# Autodesk Inventor assembly: base_ass_3
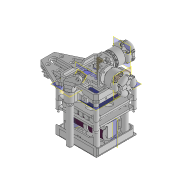
[picture p0: Inventor's stored thumbnail of the model, 180x180]
Saved by Autodesk Inventor 2020 (Build 240168000, 168)
## iProperties
Created: 2022-01-22
Part Number: base_ass_3
Document SubType Name: Assembly
Designer: Shuang Peng
Author: Shuang Peng
## Documents named in this file (18)
- D:\projects-3\soft module robot\hardware\diff module 3\base_ass_3.iam
- D:\projects-3\soft module robot\hardware\diff module 3\ext_shell_1.ipt
- D:\projects-3\soft module robot\hardware\diff module 3\brushless sub driver v1\brushless sub driver.iam
- D:\projects-3\soft module robot\hardware\diff module 3\pin_2_40.ipt
- D:\projects-3\soft module robot\hardware\diff module 3\ext_shell_2.ipt
- D:\projects-3\soft module robot\hardware\diff module 3\bridge_linker_1.ipt
- D:\projects-3\soft module robot\hardware\diff module 3\ext_shell_3.ipt
- D:\projects-3\soft module robot\hardware\diff module 3\bat_pack.iam
- D:\projects-3\soft module robot\hardware\diff module 3\ext_shell_top.ipt
- D:\projects-3\soft module robot\hardware\diff module 3\balancing_wheel_1.ipt
- D:\projects-3\soft module robot\hardware\diff module 3\balancing_wheel_2.ipt
- D:\projects-3\soft module robot\hardware\diff module 3\pin_6_40.ipt
- D:\projects-3\soft module robot\hardware\diff module 3\bearing_3_6_2.ipt
- D:\projects-3\soft module robot\hardware\diff module 3\c_roller_1.ipt
- D:\projects-3\soft module robot\hardware\diff module 3\tag.ipt
- D:\projects-3\soft module robot\hardware\diff module 3\wheel_pin_1.ipt
- D:\projects-3\soft module robot\hardware\diff module 3\pin_3_6.ipt
- D:\projects-3\soft module robot\hardware\diff module 3\2sr_ass_tmp.iam
## Components (27 placed, 17 different names)
1. ext_shell_1:1 — Mate:2, Flush:8, Insert:3, Insert:4, Insert:5, Insert:6, Insert:7, Insert:8, Flush:9, Flush:10, Insert:9, Insert:10, Flush:15, Insert:11, Insert:12, Mate:7, Insert:25, Insert:26
2. brushless sub driver:1 [sub-assembly] — Mate:2, Flush:8
3. pin_2_40:1 — Insert:3
4. pin_2_40:2 — Insert:5
5. pin_2_40:3 — Insert:6
6. pin_2_40:4 — Insert:4
7. ext_shell_2:1 — Insert:7, Insert:8, Flush:11, Tangent:6, Tangent:7, Flush:22, Tangent:8, Tangent:9, Tangent:10, Tangent:11, Tangent:12, Insert:23, Insert:24
8. bridge_linker_1:1 — Flush:9, Flush:10, Insert:9, Insert:10
9. ext_shell_3:1 — Flush:11, Mate:3, Flush:12, Flush:13, Flush:14, Insert:21, Insert:22, Insert:23, Insert:24
10. bat_pack:1 [sub-assembly] — Mate:3, Flush:12, Flush:13
11. ext_shell_top:1 — Flush:14, Mate:5, Flush:24, Mate:6, Insert:21, Insert:22
12. balancing_wheel_1:1 — Flush:15, Insert:11, Insert:12, Insert:13, Insert:15, Insert:16
13. balancing_wheel_2:1 — Insert:13, Insert:17
14. pin_6_40:1 — Flush:21, Tangent:5, Tangent:7, Tangent:12
15. pin_6_40:2 — Flush:20, Tangent:4, Tangent:5, Tangent:11
16. pin_6_40:3 — Flush:19, Tangent:3, Tangent:4, Tangent:10
17. pin_6_40:4 — Flush:18, Tangent:2, Tangent:3, Tangent:9
18. pin_6_40:5 — Flush:17, Tangent:1, Tangent:2, Tangent:8
19. pin_6_40:6 — Flush:17, Flush:18, Flush:19, Flush:20, Flush:21, Tangent:1, Tangent:6, Flush:22
20. bearing_3_6_2:1 — Insert:16
21. bearing_3_6_2:2 — Insert:15, Insert:19
22. bearing_3_6_2:3 — Insert:17, Insert:18, Insert:20
23. c_roller_1:1 — Insert:18
24. tag:1 — Mate:5, Flush:24, Mate:6
25. wheel_pin_1:1 — Insert:19
26. pin_3_6:1 — Insert:20
27. 2sr_ass_tmp:1 [sub-assembly] — Mate:7, Insert:25, Insert:26
## Relationships (55: Insert 23, Flush 15, Tangent 12, Mate 5)
- Mate:2 (4 mm): ext_shell_1:1 ↔ brushless sub driver:1
- Flush:8 (1.5 mm): ext_shell_1:1 ↔ brushless sub driver:1
- Insert:3: ext_shell_1:1 ↔ pin_2_40:1
- Insert:4: ext_shell_1:1 ↔ pin_2_40:4
- Insert:5: ext_shell_1:1 ↔ pin_2_40:2
- Insert:6: ext_shell_1:1 ↔ pin_2_40:3
- Insert:7 (3 mm): ext_shell_1:1 ↔ ext_shell_2:1
- Insert:8 (3 mm): ext_shell_1:1 ↔ ext_shell_2:1
- Flush:9: ext_shell_1:1 ↔ bridge_linker_1:1
- Flush:10: ext_shell_1:1 ↔ bridge_linker_1:1
- Insert:9: ext_shell_1:1 ↔ bridge_linker_1:1
- Insert:10: ext_shell_1:1 ↔ bridge_linker_1:1
- Flush:11: ext_shell_2:1 ↔ ext_shell_3:1
- Mate:3 (1 mm): ext_shell_3:1 ↔ bat_pack:1
- Flush:12 (12 mm): ext_shell_3:1 ↔ bat_pack:1
- Flush:13: ext_shell_3:1 ↔ bat_pack:1
- Flush:14: ext_shell_3:1 ↔ ext_shell_top:1
- Flush:15: ext_shell_1:1 ↔ balancing_wheel_1:1
- Insert:11: ext_shell_1:1 ↔ balancing_wheel_1:1
- Insert:12: ext_shell_1:1 ↔ balancing_wheel_1:1
- Insert:13: balancing_wheel_1:1 ↔ balancing_wheel_2:1
- Flush:17: pin_6_40:5 ↔ pin_6_40:6
- Flush:18: pin_6_40:4 ↔ pin_6_40:6
- Flush:19: pin_6_40:3 ↔ pin_6_40:6
- Flush:20: pin_6_40:2 ↔ pin_6_40:6
- Flush:21: pin_6_40:1 ↔ pin_6_40:6
- Tangent:1: pin_6_40:5 ↔ pin_6_40:6
- Tangent:2: pin_6_40:4 ↔ pin_6_40:5
- Tangent:3: pin_6_40:3 ↔ pin_6_40:4
- Tangent:4: pin_6_40:2 ↔ pin_6_40:3
- Tangent:5: pin_6_40:1 ↔ pin_6_40:2
- Tangent:6: ext_shell_2:1 ↔ pin_6_40:6
- Tangent:7: ext_shell_2:1 ↔ pin_6_40:1
- Flush:22 (1 mm): ext_shell_2:1 ↔ pin_6_40:6
- Tangent:8: ext_shell_2:1 ↔ pin_6_40:5
- Tangent:9: ext_shell_2:1 ↔ pin_6_40:4
- Tangent:10: ext_shell_2:1 ↔ pin_6_40:3
- Tangent:11: ext_shell_2:1 ↔ pin_6_40:2
- Tangent:12: ext_shell_2:1 ↔ pin_6_40:1
- Insert:15: balancing_wheel_1:1 ↔ bearing_3_6_2:2
- Insert:16: balancing_wheel_1:1 ↔ bearing_3_6_2:1
- Insert:17: balancing_wheel_2:1 ↔ bearing_3_6_2:3
- Insert:18: bearing_3_6_2:3 ↔ c_roller_1:1
- Mate:5: ext_shell_top:1 ↔ tag:1
- Flush:24 (-0.5 mm): ext_shell_top:1 ↔ tag:1
- Mate:6 (0.5 mm): ext_shell_top:1 ↔ tag:1
- Insert:19 (-6 mm): bearing_3_6_2:2 ↔ wheel_pin_1:1
- Insert:20 (0.5 mm): bearing_3_6_2:3 ↔ pin_3_6:1
- Insert:21: ext_shell_3:1 ↔ ext_shell_top:1
- Insert:22: ext_shell_3:1 ↔ ext_shell_top:1
- Insert:23: ext_shell_2:1 ↔ ext_shell_3:1
- Insert:24: ext_shell_2:1 ↔ ext_shell_3:1
- Mate:7: ext_shell_1:1 ↔ 2sr_ass_tmp:1
- Insert:25: ext_shell_1:1 ↔ 2sr_ass_tmp:1
- Insert:26: ext_shell_1:1 ↔ 2sr_ass_tmp:1
